# Autodesk Inventor assembly: Boden
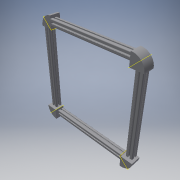
[picture p0: Inventor's stored thumbnail of the model, 180x180]
Saved by Autodesk Inventor 2019 (Build 230136000, 136)
## iProperties
Created: 2018-08-15
Part Number: Boden
Document SubType Name: Assembly
Designer: Julia
Author: Julia
## Documents named in this file (3)
- C:\Users\Julia\Documents\Inventor\3D_Drucker_v01\Boden.iam
- C:\Users\Julia\Documents\Inventor\3D_Drucker_v01\Boden_Ecke.iam
- C:\Users\Julia\Documents\Inventor\3D_Drucker_v01\Alu_Proil_40.ipt
## Components (8 placed, 2 different names)
1. Boden_Ecke:1 [sub-assembly] — Mate:1, Mate:2, Angle:2, Mate:14, Angle:6, Mate:15
2. Boden_Ecke:2 [sub-assembly] — Mate:3, Mate:4, Mate:5, Mate:6, Angle:1, Mate:13
3. Boden_Ecke:3 [sub-assembly] — Mate:7, Angle:3, Mate:8, Mate:9, Mate:10, Angle:4
4. Boden_Ecke:4 [sub-assembly] — Mate:11, Mate:12, Angle:5
5. Alu_Proil_40:1 — Mate:1, Mate:2, Mate:3, Mate:4, Angle:2
6. Alu_Proil_40:2 — Mate:5, Mate:6, Angle:1, Mate:7, Angle:3, Mate:8, Mate:13
7. Alu_Proil_40:3 — Mate:9, Mate:10, Angle:4, Mate:11, Mate:12, Angle:5
8. Alu_Proil_40:4 — Mate:14, Angle:6, Mate:15
## Relationships (21: Mate 15, Angle 6)
- Mate:1: Boden_Ecke:1 ↔ Alu_Proil_40:1
- Mate:2: Boden_Ecke:1 ↔ Alu_Proil_40:1
- Mate:3: Boden_Ecke:2 ↔ Alu_Proil_40:1
- Mate:4: Boden_Ecke:2 ↔ Alu_Proil_40:1
- Mate:5: Boden_Ecke:2 ↔ Alu_Proil_40:2
- Mate:6: Boden_Ecke:2 ↔ Alu_Proil_40:2
- Angle:1 (0 deg): Boden_Ecke:2 ↔ Alu_Proil_40:2
- Angle:2 (0 deg): Boden_Ecke:1 ↔ Alu_Proil_40:1
- Mate:7: Boden_Ecke:3 ↔ Alu_Proil_40:2
- Angle:3 (0 deg): Boden_Ecke:3 ↔ Alu_Proil_40:2
- Mate:8: Boden_Ecke:3 ↔ Alu_Proil_40:2
- Mate:9: Boden_Ecke:3 ↔ Alu_Proil_40:3
- Mate:10: Boden_Ecke:3 ↔ Alu_Proil_40:3
- Angle:4 (0 deg): Boden_Ecke:3 ↔ Alu_Proil_40:3
- Mate:11: Boden_Ecke:4 ↔ Alu_Proil_40:3
- Mate:12: Boden_Ecke:4 ↔ Alu_Proil_40:3
- Angle:5 (0 deg): Boden_Ecke:4 ↔ Alu_Proil_40:3
- Mate:13: Boden_Ecke:2 ↔ Alu_Proil_40:2
- Mate:14: Boden_Ecke:1 ↔ Alu_Proil_40:4
- Angle:6 (0 deg): Boden_Ecke:1 ↔ Alu_Proil_40:4
- Mate:15: Boden_Ecke:1 ↔ Alu_Proil_40:4
